# Autodesk Inventor assembly: ASY ДМФ 0100 Барабан v2.1
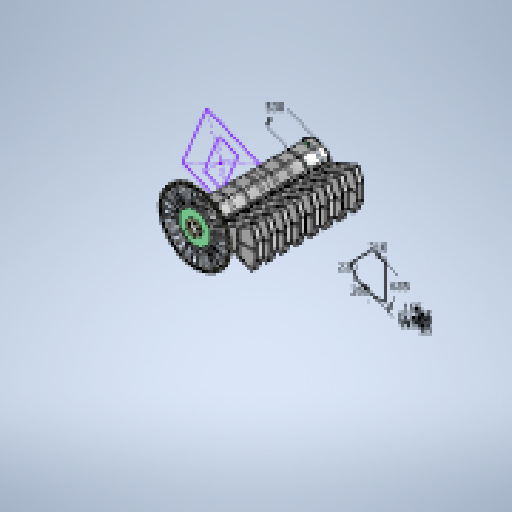
[picture p0: Inventor's stored thumbnail of the model, 512x512]
Saved by Autodesk Inventor 2026.2 (Build 302298010, 298A)
## iProperties
Created: 2024-04-28
Part Number: ASY ДМФ 0100 Барабан v2.1
Document SubType Name: Assembly
Designer: pokla
Author: pokla
## Documents named in this file (15)
- C:\Users\admin\Documents\Inventor\DMF-Disk-Micro-Filter\Барабан v2.1\ASY ДМФ 0100 Барабан v2.1.iam
- C:\Users\admin\Documents\Inventor\DMF-Disk-Micro-Filter\Барабан v2.1\DMF 01 21 Барабан торец НОС v2.1.ipt
- C:\Users\admin\Documents\Inventor\DMF-Disk-Micro-Filter\Барабан v2.1\DMF 01 13 Барабан Лист лев брт v2.1.ipt
- C:\Users\admin\Documents\Inventor\DMF-Disk-Micro-Filter\Барабан v2.1\DMF 01 14 Барабан Лист прав брт v2.1.ipt
- C:\Users\admin\Documents\Inventor\DMF-Disk-Micro-Filter\Барабан v2.1\DMF 01 31 Барабан Опорное кольцо НОС v2.1.ipt
- C:\Users\admin\Documents\Inventor\DMF-Disk-Micro-Filter\Барабан v2.1\DMF 01 17 опора крышки v2.1.ipt
- C:\Users\admin\Documents\Inventor\DMF-Disk-Micro-Filter\Барабан v2.1\DMF 000 размеры v2.1.ipt
- C:\Users\admin\Documents\Inventor\DMF-Disk-Micro-Filter\Барабан v2.1\ASY DMF 010 cap v2.1.iam
- C:\Users\admin\Documents\Inventor\DMF-Disk-Micro-Filter\Барабан v2.1\DMF 01 32 Барабан Опорное кольцо КОРМА v2.1.ipt
- C:\Users\admin\Documents\Inventor\DMF-Disk-Micro-Filter\Барабан v2.1\DMF 01 22 Барабан торец КОРМА v2.1.ipt
- C:\Users\admin\Documents\Inventor\DMF-Disk-Micro-Filter\Барабан v2.1\ASY DMF filter package v2.1.iam
- C:\Users\admin\Documents\Inventor\DMF-Disk-Micro-Filter\Барабан v2.1\DMF 01 11 cylinder sheet cap v2.1.ipt
- C:\Users\admin\Documents\Inventor\DMF-Disk-Micro-Filter\ContentCenter\en-US\DIN 913\DIN 913 - M12 x 20.ipt
- C:\Users\admin\Documents\Inventor\DMF-Disk-Micro-Filter\Барабан v2.1\DMF 01 11 cylinder sheet cap v2.1_CPY.ipt
- C:\Users\admin\Documents\Inventor\DMF-Disk-Micro-Filter\Барабан v2.1\ASY DMF 01 20 snout.iam
## Components (29 placed, 19 different names)
1. DMF 000 размеры v2.1.ipt:1
2. DMF 01 21 Барабан торец НОС v2.1.ipt:1 — Rigid:115
3. DMF 01 31 Барабан Опорное кольцо НОС v2.1.ipt:1
4. DMF 01 32 Барабан Опорное кольцо КОРМА v2.1.ipt:1 — Rigid:126
5. DMF 01 22 Барабан торец КОРМА v2.1.ipt:1 — Rigid:51, Mate:37, Rigid:97, Mate:46, Mate:50, Flush:36, Mate:51, Rigid:126, Mate:54
6. DMF 01 13 Барабан Лист лев брт v2.1.ipt:1 — Rigid:51, Rigid:98
7. DMF 01 14 Барабан Лист прав брт v2.1.ipt:1 — Mate:54, Mate:55, Mate:56
8. DMF 01 17 опора крышки v2.1.ipt:1 — Mate:37, Mate:46, Mate:47, Mate:48, Rigid:112
9. DMF 01 11 cylinder sheet cap v2.1.ipt:1 — Mate:47, Rotational:1, Rigid:122, Mate:55, Mate:56
10. DMF 01 13 Барабан Лист лев брт v2.1:2 — Rigid:97, Rigid:99, Mate:48
11. DMF 01 13 Барабан Лист лев брт v2.1:3 — Rigid:98
12. DMF 01 13 Барабан Лист лев брт v2.1:4 — Rigid:99, Rigid:115
13. DMF 01 17 опора крышки v2.1:4 — Rigid:112
14. DIN 913 M12 x 20:1 — Rotational:1
15. DMF 01 11 cylinder sheet cap v2.1:2 — Rigid:122, Rigid:123
16. DMF 01 11 cylinder sheet cap v2.1_CPY:1 — Rigid:123
17. ASY DMF 010 cap v2.1.iam:1 [sub-assembly]
18. ASY DMF 010 cap v2.1:2 [sub-assembly]
19. ASY DMF 010 cap v2.1:3 [sub-assembly]
20. ASY DMF 010 cap v2.1:4 [sub-assembly]
21. ASY DMF 01 20 snout:1 [sub-assembly]
22. ASY DMF filter package v2.1.iam:1 [sub-assembly]
23. ASY DMF filter package v2.1:2 [sub-assembly]
24. ASY DMF filter package v2.1:3 [sub-assembly]
25. ASY DMF filter package v2.1:4 [sub-assembly]
26. ASY DMF filter package v2.1:5 [sub-assembly]
27. ASY DMF filter package v2.1:6 [sub-assembly]
28. ASY DMF filter package v2.1:7 [sub-assembly]
29. ASY DMF filter package v2.1:8 [sub-assembly]
## Component patterns: (8 elements, first: ASY DMF filter package v2.1.iam:1)
## Relationships (32: WeldJoint 15, Mate 12, Flush 4, RevoluteJoint 1)
- Rigid:51 [WeldJoint]: DMF 01 22 Барабан торец КОРМА v2.1.ipt:1 ↔ DMF 01 13 Барабан Лист лев брт v2.1.ipt:1
- Mate:37: DMF 01 22 Барабан торец КОРМА v2.1.ipt:1 ↔ DMF 01 17 опора крышки v2.1.ipt:1
- [Mate]: DMF 01 22 Барабан торец КОРМА v2.1.ipt:1 ↔ DMF 01 11 cylinder sheet cap v2.1.ipt:1
- [Flush]: DMF 01 22 Барабан торец КОРМА v2.1.ipt:1 ↔ DMF 01 11 cylinder sheet cap v2.1.ipt:1
- [Flush]: DMF 01 22 Барабан торец КОРМА v2.1.ipt:1 ↔ DMF 01 11 cylinder sheet cap v2.1.ipt:1
- [WeldJoint]: DMF 01 11 cylinder sheet cap v2.1.ipt:1 ↔ ASY DMF filter package v2.1.iam:1
- Rigid:97 [WeldJoint]: DMF 01 22 Барабан торец КОРМА v2.1.ipt:1 ↔ DMF 01 13 Барабан Лист лев брт v2.1:2
- Rigid:98 [WeldJoint]: DMF 01 13 Барабан Лист лев брт v2.1.ipt:1 ↔ DMF 01 13 Барабан Лист лев брт v2.1:3
- Rigid:99 [WeldJoint]: DMF 01 13 Барабан Лист лев брт v2.1:2 ↔ DMF 01 13 Барабан Лист лев брт v2.1:4
- Mate:46: DMF 01 22 Барабан торец КОРМА v2.1.ipt:1 ↔ DMF 01 17 опора крышки v2.1.ipt:1
- Mate:47: DMF 01 17 опора крышки v2.1.ipt:1 ↔ DMF 01 11 cylinder sheet cap v2.1.ipt:1
- Mate:48: DMF 01 17 опора крышки v2.1.ipt:1 ↔ DMF 01 13 Барабан Лист лев брт v2.1:2
- Rigid:112 [WeldJoint]: DMF 01 17 опора крышки v2.1.ipt:1 ↔ DMF 01 17 опора крышки v2.1:4
- Mate:50: DMF 01 22 Барабан торец КОРМА v2.1.ipt:1
- Flush:36: DMF 01 22 Барабан торец КОРМА v2.1.ipt:1
- Mate:51: DMF 01 22 Барабан торец КОРМА v2.1.ipt:1
- Rigid:115 [WeldJoint]: DMF 01 21 Барабан торец НОС v2.1.ipt:1 ↔ DMF 01 13 Барабан Лист лев брт v2.1:4
- [WeldJoint]: DMF 01 21 Барабан торец НОС v2.1.ipt:1 ↔ ASY DMF 01 20 snout:1
- Rotational:1 [RevoluteJoint]: DMF 01 11 cylinder sheet cap v2.1.ipt:1 ↔ DIN 913 M12 x 20:1
- Rigid:122 [WeldJoint]: DMF 01 11 cylinder sheet cap v2.1.ipt:1 ↔ DMF 01 11 cylinder sheet cap v2.1:2
- Rigid:123 [WeldJoint]: DMF 01 11 cylinder sheet cap v2.1:2 ↔ DMF 01 11 cylinder sheet cap v2.1_CPY:1
- Rigid:126 [WeldJoint]: DMF 01 32 Барабан Опорное кольцо КОРМА v2.1.ipt:1 ↔ DMF 01 22 Барабан торец КОРМА v2.1.ipt:1
- Mate:54: DMF 01 22 Барабан торец КОРМА v2.1.ipt:1 ↔ DMF 01 14 Барабан Лист прав брт v2.1.ipt:1
- Mate:55: DMF 01 14 Барабан Лист прав брт v2.1.ipt:1 ↔ DMF 01 11 cylinder sheet cap v2.1.ipt:1
- Mate:56: DMF 01 14 Барабан Лист прав брт v2.1.ipt:1 ↔ DMF 01 11 cylinder sheet cap v2.1.ipt:1
- [Mate]: ASY DMF 010 cap v2.1.iam:1 ↔ ASY DMF 01 20 snout:1
- [Mate]: ASY DMF 010 cap v2.1.iam:1 ↔ ASY DMF 01 20 snout:1
- [Flush]: ASY DMF 010 cap v2.1.iam:1 ↔ ASY DMF 01 20 snout:1
- [WeldJoint]: ASY DMF 010 cap v2.1:2 ↔ ASY DMF 01 20 snout:1
- [WeldJoint]: ASY DMF 010 cap v2.1:3 ↔ ASY DMF 01 20 snout:1
- [WeldJoint]: ASY DMF 010 cap v2.1:4 ↔ ASY DMF 01 20 snout:1
- [WeldJoint]: DMF 01 31 Барабан Опорное кольцо НОС v2.1.ipt:1 ↔ ASY DMF 01 20 snout:1
